# Autodesk Inventor assembly: Table_Setup
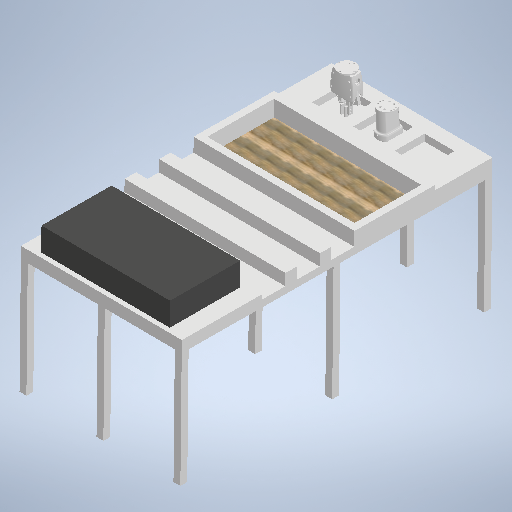
[picture p0: Inventor's stored thumbnail of the model, 512x512]
Saved by Autodesk Inventor 2025 (Build 290162000, 162)
## iProperties
Created: 2024-06-19
Part Number: Table_Setup
Document SubType Name: Assembly
Designer: User
Author: User
## Documents named in this file (5)
- C:\Users\User\OneDrive\Documents\FYP\Inventor_Designs\Setups\Table_Setup.iam
- C:\Users\User\OneDrive\Documents\FYP\Inventor_Designs\Platform\Table.ipt
- C:\Users\User\OneDrive\Documents\FYP\Inventor_Designs\Grippers\Gripper.ipt
- C:\Users\User\OneDrive\Documents\FYP\Inventor_Designs\Grippers\Vacuum Gripper.ipt
- C:\Users\User\OneDrive\Documents\FYP\Inventor_Designs\Platform\Blackout Box.ipt
## Components (4 placed, 4 different names)
1. Table:1 — Mate:1, Mate:2, Mate:4
2. Gripper:1 — Mate:2
3. Vacuum Gripper:1 — Mate:1
4. Blackout Box:1 — Mate:4
## Relationships (3: Mate 3)
- Mate:1: Table:1 ↔ Vacuum Gripper:1
- Mate:2: Table:1 ↔ Gripper:1
- Mate:4: Table:1 ↔ Blackout Box:1
